# Autodesk Inventor assembly: ENSAMBLE MECANISMO DE INGRESO
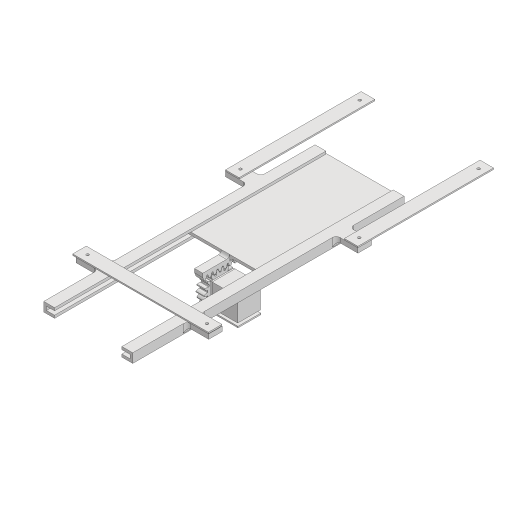
[picture p0: Inventor's stored thumbnail of the model, 512x512]
Saved by Autodesk Inventor 2024 (Build 280153000, 153)
## iProperties
Created: 2024-06-13
Part Number: ENSAMBLE MECANISMO DE INGRESO
Document SubType Name: Assembly
Designer: Jhuliams
Author: Jhuliams
## Documents named in this file (7)
- C:\Users\Jhuliams\Documents\GitHub\RECICLADOR_MODELO_3D\MECANISMO DE COMPACTADO\ENSAMBLE MECANISMO DE INGRESO.iam
- C:\Users\Jhuliams\Documents\GitHub\RECICLADOR_MODELO_3D\MECANISMO DE COMPACTADO\PINON DE TAPA PRINCIPAL.ipt
- C:\Users\Jhuliams\Documents\GitHub\RECICLADOR_MODELO_3D\MECANISMO DE COMPACTADO\TAPA PRICIPAL CON CREMALLERA.ipt
- C:\Users\Jhuliams\Documents\GitHub\RECICLADOR_MODELO_3D\MECANISMO DE COMPACTADO\GUIA DE TAPA PRINCIPAL.ipt
- C:\Users\Jhuliams\Documents\GitHub\RECICLADOR_MODELO_3D\MECANISMO DE COMPACTADO\NEMA 17 PARA TAPA PRINCIPAL.ipt
- C:\Users\Jhuliams\Documents\GitHub\RECICLADOR_MODELO_3D\MECANISMO DE COMPACTADO\SOPORTE DE NEMA.ipt
- C:\Users\Jhuliams\Documents\GitHub\RECICLADOR_MODELO_3D\MECANISMO DE COMPACTADO\PLETINA PARA CARA INCLINADA.ipt
## Components (9 placed, 6 different names)
1. PINON DE TAPA PRINCIPAL:1 — Mate:1, Flush:1, Flush:2, Rotation/Translation:1, Mate:7, Mate:8
2. TAPA PRICIPAL CON CREMALLERA:1 — Flush:2, Mate:2, Rotation/Translation:1, Mate:3, Mate:6, Mate:9, Mate:12, Mate:13
3. GUIA DE TAPA PRINCIPAL:1 — Mate:3, Mate:6, Flush:8, Flush:9, Flush:11, Mate:16, Flush:13
4. NEMA 17 PARA TAPA PRINCIPAL:1 — Mate:7, Mate:8, Mate:9, Mate:10, Mate:11, Flush:8, Flush:15
5. SOPORTE DE NEMA:1 — Mate:10, Mate:11, Flush:15
6. GUIA DE TAPA PRINCIPAL:2 — Mate:12, Flush:9, Mate:13, Flush:10, Mate:14, Flush:12, Mate:15, Flush:14
7. PLETINA PARA CARA INCLINADA:1 — Flush:10, Mate:14
8. PLETINA PARA CARA INCLINADA:2 — Flush:12, Mate:15, Flush:14
9. PLETINA PARA CARA INCLINADA:3 — Flush:11, Mate:16, Flush:13
## Relationships (26: Mate 14, Flush 11, RelateRotateTranslate 1)
- Mate:1: PINON DE TAPA PRINCIPAL:1
- Flush:1: PINON DE TAPA PRINCIPAL:1
- Flush:2: PINON DE TAPA PRINCIPAL:1 ↔ TAPA PRICIPAL CON CREMALLERA:1
- Flush:4 (27 mm)
- Mate:2 (3.75 mm): TAPA PRICIPAL CON CREMALLERA:1
- Rotation/Translation:1 [RelateRotateTranslate] (169.646 mm): PINON DE TAPA PRINCIPAL:1 ↔ TAPA PRICIPAL CON CREMALLERA:1
- Mate:3 (2 mm): TAPA PRICIPAL CON CREMALLERA:1 ↔ GUIA DE TAPA PRINCIPAL:1
- Mate:6: TAPA PRICIPAL CON CREMALLERA:1 ↔ GUIA DE TAPA PRINCIPAL:1
- Mate:7: PINON DE TAPA PRINCIPAL:1 ↔ NEMA 17 PARA TAPA PRINCIPAL:1
- Mate:8 (6 mm): PINON DE TAPA PRINCIPAL:1 ↔ NEMA 17 PARA TAPA PRINCIPAL:1
- Mate:9 (9.75 mm): TAPA PRICIPAL CON CREMALLERA:1 ↔ NEMA 17 PARA TAPA PRINCIPAL:1
- Mate:10: NEMA 17 PARA TAPA PRINCIPAL:1 ↔ SOPORTE DE NEMA:1
- Mate:11: NEMA 17 PARA TAPA PRINCIPAL:1 ↔ SOPORTE DE NEMA:1
- Flush:8 (-215 mm): GUIA DE TAPA PRINCIPAL:1 ↔ NEMA 17 PARA TAPA PRINCIPAL:1
- Mate:12: TAPA PRICIPAL CON CREMALLERA:1 ↔ GUIA DE TAPA PRINCIPAL:2
- Flush:9: GUIA DE TAPA PRINCIPAL:1 ↔ GUIA DE TAPA PRINCIPAL:2
- Mate:13 (2 mm): TAPA PRICIPAL CON CREMALLERA:1 ↔ GUIA DE TAPA PRINCIPAL:2
- Flush:10: GUIA DE TAPA PRINCIPAL:2 ↔ PLETINA PARA CARA INCLINADA:1
- Mate:14: GUIA DE TAPA PRINCIPAL:2 ↔ PLETINA PARA CARA INCLINADA:1
- Flush:11: GUIA DE TAPA PRINCIPAL:1 ↔ PLETINA PARA CARA INCLINADA:3
- Flush:12: GUIA DE TAPA PRINCIPAL:2 ↔ PLETINA PARA CARA INCLINADA:2
- Mate:15: GUIA DE TAPA PRINCIPAL:2 ↔ PLETINA PARA CARA INCLINADA:2
- Mate:16: GUIA DE TAPA PRINCIPAL:1 ↔ PLETINA PARA CARA INCLINADA:3
- Flush:13: GUIA DE TAPA PRINCIPAL:1 ↔ PLETINA PARA CARA INCLINADA:3
- Flush:14: GUIA DE TAPA PRINCIPAL:2 ↔ PLETINA PARA CARA INCLINADA:2
- Flush:15: NEMA 17 PARA TAPA PRINCIPAL:1 ↔ SOPORTE DE NEMA:1
